# Autodesk Inventor assembly: Arm
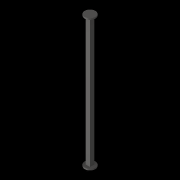
[picture p0: Inventor's stored thumbnail of the model, 180x180]
Saved by Autodesk Inventor 2019 (Build 230136000, 136)
## iProperties
Created: 2018-12-30
Part Number: Arm
Document SubType Name: Assembly
Designer: JedrzejDankowski
Author: JedrzejDankowski
## Documents named in this file (2)
- C:\Users\MJ\Documents\AiFit-Inventor\Arm.iam
- C:\Users\MJ\Documents\AiFit-Inventor\guide.ipt
## Components (1 placed, 1 different names)
1. guide:1 — Mate:4, Mate:5, Flush:1
## Relationships (3: Mate 2, Flush 1)
- Mate:4: guide:1
- Mate:5: guide:1
- Flush:1: guide:1
